# Autodesk Inventor assembly: Montagem peças internas
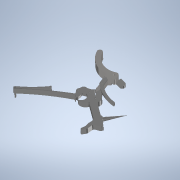
[picture p0: Inventor's stored thumbnail of the model, 180x180]
Saved by Autodesk Inventor 2021 (Build 250183000, 183)
## iProperties
Created: 2020-11-29
Part Number: Montagem peças internas
Document SubType Name: Assembly
Designer: Bruno
Author: Bruno
## Documents named in this file (11)
- C:\Users\Bruno\Documents\Quadirmestre Suplementar\Projeto Assistido por Computador\Novas peças revólver\Montagem peças internas.iam
- C:\Users\Bruno\Documents\Quadirmestre Suplementar\Projeto Assistido por Computador\Novas peças revólver\Part28.ipt
- C:\Users\Bruno\Documents\Quadirmestre Suplementar\Projeto Assistido por Computador\Novas peças revólver\Part28_2.ipt
- C:\Users\Bruno\Documents\Quadirmestre Suplementar\Projeto Assistido por Computador\Novas peças revólver\Part29.ipt
- C:\Users\Bruno\Documents\Quadirmestre Suplementar\Projeto Assistido por Computador\Novas peças revólver\Part33.ipt
- C:\Users\Bruno\Documents\Quadirmestre Suplementar\Projeto Assistido por Computador\Novas peças revólver\Coil_28_31.ipt
- C:\Users\Bruno\Documents\Quadirmestre Suplementar\Projeto Assistido por Computador\Novas peças revólver\Part38.ipt
- C:\Users\Bruno\Documents\Quadirmestre Suplementar\Projeto Assistido por Computador\Novas peças revólver\Part43.ipt
- C:\Users\Bruno\Documents\Quadirmestre Suplementar\Projeto Assistido por Computador\Novas peças revólver\Placa gatilho.ipt
- C:\Users\Bruno\Documents\Quadirmestre Suplementar\Projeto Assistido por Computador\Novas peças revólver\Parte98.ipt
- C:\Users\Bruno\Documents\Quadirmestre Suplementar\Projeto Assistido por Computador\Novas peças revólver\Part59.ipt
## Components (10 placed, 10 different names)
1. Part28:1 — Mate:18, Flush:3, Rígida:1, Coincidente:27, Alinhado:4
2. Part28_2:1 — Coincidente:5, Coincidente:6, Rígida:1, Alinhado:5, Coincidente:28
3. Part29:1 — Coincidente:27, Alinhado:4
4. Part33:1 — Coincidente:5, Coincidente:6, Coincidente:8, Coincidente:9
5. Coil_28_31:1 — Mate:18, Flush:3
6. Part38:1 — Coincidente:8, Coincidente:9
7. Part43:1 — Mate:23, Mate:24, Rotational:1, Alinhado:5, Coincidente:28, Coincidente:29, Coincidente:30
8. Placa gatilho:1 — Mate:23, Mate:24
9. Parte98:1 — Rotational:1, Coincidente:31
10. Part59:1 — Coincidente:29, Coincidente:30
## Relationships (17: Mate 12, Flush 3, RevoluteJoint 1, WeldJoint 1)
- Coincidente:5 [Mate]: Part28_2:1 ↔ Part33:1
- Coincidente:6 [Mate]: Part28_2:1 ↔ Part33:1
- Coincidente:8 [Mate]: Part33:1 ↔ Part38:1
- Coincidente:9 [Mate]: Part33:1 ↔ Part38:1
- Mate:18: Part28:1 ↔ Coil_28_31:1
- Flush:3 (-0.05 mm): Part28:1 ↔ Coil_28_31:1
- Mate:23: Part43:1 ↔ Placa gatilho:1
- Mate:24: Part43:1 ↔ Placa gatilho:1
- Rotational:1 [RevoluteJoint]: Part43:1 ↔ Parte98:1
- Rígida:1 [WeldJoint]: Part28:1 ↔ Part28_2:1
- Coincidente:27 [Mate]: Part28:1 ↔ Part29:1
- Alinhado:4 [Flush]: Part28:1 ↔ Part29:1
- Alinhado:5 [Flush]: Part28_2:1 ↔ Part43:1
- Coincidente:28 [Mate]: Part28_2:1 ↔ Part43:1
- Coincidente:29 [Mate]: Part43:1 ↔ Part59:1
- Coincidente:30 [Mate]: Part43:1 ↔ Part59:1
- Coincidente:31 [Mate]: Parte98:1
